# Autodesk Inventor assembly: Scissor Lift
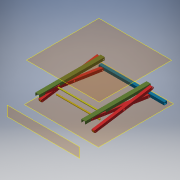
[picture p0: Inventor's stored thumbnail of the model, 180x180]
Saved by Autodesk Inventor 2017 SP1 (Build 210196100, 196)
## iProperties
Created: 2018-01-12
Part Number: Scissor Lift
Document SubType Name: Assembly
Designer: Ben
Author: Ben
## Documents named in this file (6)
- C:\Users\Ben\Desktop\Projects\2018 Robot\Scissor Lift\Scissor Lift.iam
- C:\Users\Ben\Desktop\Projects\2018 Robot\Scissor Lift\Front lift arm.ipt
- C:\Users\Ben\Desktop\Projects\2018 Robot\Scissor Lift\lift wheel.ipt
- C:\Users\Ben\Desktop\Projects\2018 Robot\Scissor Lift\lift rails.ipt
- C:\Users\Ben\Desktop\Projects\2018 Robot\Scissor Lift\lift support arm.ipt
- C:\Users\Ben\Desktop\Projects\2018 Robot\Scissor Lift\cross support.ipt
## Components (13 placed, 5 different names)
1. Front lift arm:1 — Insert:6, Mate:4, Insert:8, Flush:14, Mate:11, Flush:17, Insert:9
2. Front lift arm:2 — Insert:5, Insert:7, Mate:4, Mate:9, Flush:17, Mate:13, Mate:14, Insert:10
3. Front lift arm:3 — Flush:9, Insert:4, Insert:8, Mate:17
4. Front lift arm:4 — Flush:9, Insert:3, Insert:7, Mate:16
5. lift wheel:1 — Insert:3, Tangent:1
6. lift wheel:2 — Insert:4, Tangent:2
7. lift wheel:3 — Insert:6, Tangent:4
8. lift wheel:4 — Insert:5, Tangent:3
9. lift rails:1 — Tangent:4, Mate:11, Mate:17
10. lift rails:2 — Tangent:3, Mate:9, Mate:16
11. lift support arm:1 — Mate:6, Mate:7, Flush:14, Mate:14
12. cross support:1 — Insert:9, Insert:10
13. cross support:2
## Relationships (26: Mate 9, Insert 8, Flush 5, Tangent 4)
- Flush:9: Front lift arm:3 ↔ Front lift arm:4
- Insert:3 (1.5875 mm): Front lift arm:4 ↔ lift wheel:1
- Insert:4 (1.5875 mm): Front lift arm:3 ↔ lift wheel:2
- Insert:5 (1.5875 mm): Front lift arm:2 ↔ lift wheel:4
- Insert:6 (1.5875 mm): Front lift arm:1 ↔ lift wheel:3
- Insert:7 (6.35 mm): Front lift arm:2 ↔ Front lift arm:4
- Mate:4: Front lift arm:1 ↔ Front lift arm:2
- Insert:8 (6.35 mm): Front lift arm:1 ↔ Front lift arm:3
- Tangent:1: lift wheel:1
- Tangent:2: lift wheel:2
- Mate:6: lift support arm:1
- Mate:7: lift support arm:1
- Flush:14 (-25.4 mm): Front lift arm:1 ↔ lift support arm:1
- Tangent:3: lift wheel:4 ↔ lift rails:2
- Mate:9 (1.5875 mm): Front lift arm:2 ↔ lift rails:2
- Tangent:4: lift wheel:3 ↔ lift rails:1
- Mate:11 (1.5875 mm): Front lift arm:1 ↔ lift rails:1
- Flush:15 (355.6 mm)
- Flush:16 (838.2 mm)
- Flush:17: Front lift arm:1 ↔ Front lift arm:2
- Mate:13 (12.7 mm): Front lift arm:2
- Mate:14 (15.875 mm): Front lift arm:2 ↔ lift support arm:1
- Mate:16: Front lift arm:4 ↔ lift rails:2
- Mate:17: Front lift arm:3 ↔ lift rails:1
- Insert:9: Front lift arm:1 ↔ cross support:1
- Insert:10: Front lift arm:2 ↔ cross support:1
